# Autodesk Inventor assembly: Matchboxscope_VCM_v1
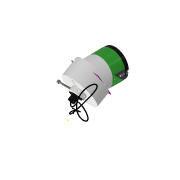
[picture p0: Inventor's stored thumbnail of the model, 180x180]
Saved by Autodesk Inventor 2022 (Build 260153000, 153)
## iProperties
Created: 2022-04-02
Part Number: Matchboxscope_VCM_v1
Document SubType Name: Assembly
Designer: Prakash Lab
Author: Prakash Lab
## Documents named in this file (13)
- C:\Users\diederichbenedict\Dropbox\Dokumente\Promotion\PROJECTS\Matchboxscope\INVENTOR\RELEASE\ESPECTROMETER\Workspace\Spectroscope_v0.iam
- C:\Users\diederichbenedict\Dropbox\Dokumente\Promotion\PROJECTS\Matchboxscope\INVENTOR\RELEASE\ESPECTROMETER\Workspace\00_ESP3-CAM.iam
- C:\Users\diederichbenedict\Dropbox\Dokumente\Promotion\PROJECTS\Matchboxscope\INVENTOR\RELEASE\ESPECTROMETER\Workspace\00_Powerbank.ipt
- C:\Users\diederichbenedict\Documents\Inventor\Content Center Files\R2022\de-DE\DIN 912\DIN 912 - M3 x 0.5 x 25 x 18.ipt
- C:\Users\diederichbenedict\Dropbox\Dokumente\Promotion\PROJECTS\Matchboxscope\INVENTOR\RELEASE\ESPECTROMETER\Workspace\Spectrometer_gratingholder_v0.ipt
- C:\Users\diederichbenedict\Dropbox\Dokumente\Promotion\PROJECTS\Matchboxscope\INVENTOR\RELEASE\ESPECTROMETER\Workspace\00_Grating_1000linesPerMM.ipt
- C:\Users\diederichbenedict\Dropbox\Dokumente\Promotion\PROJECTS\Matchboxscope\INVENTOR\RELEASE\ESPECTROMETER\Workspace\Spectrometer_pinholeholder_v0.ipt
- C:\Users\diederichbenedict\Dropbox\Dokumente\Promotion\PROJECTS\Matchboxscope\INVENTOR\RELEASE\InjectionMolded\00_mk8_nozzle_0.4STEP.ipt
- C:\Users\diederichbenedict\Dropbox\Dokumente\Promotion\PROJECTS\Matchboxscope\INVENTOR\RELEASE\ESPECTROMETER\Workspace\00_toslink_launcher_v3.ipt
- C:\Users\diederichbenedict\Dropbox\Dokumente\Promotion\PROJECTS\Matchboxscope\INVENTOR\RELEASE\ESPECTROMETER\Workspace\00_Toslink.ipt
- C:\Users\diederichbenedict\Dropbox\Dokumente\Promotion\PROJECTS\Matchboxscope\INVENTOR\RELEASE\InjectionMolded\IM_Matchboxscope_base.ipt
- C:\Users\diederichbenedict\Dropbox\Dokumente\Promotion\PROJECTS\Matchboxscope\INVENTOR\RELEASE\InjectionMolded\IM_Matchboxscope_plate.ipt
- C:\Users\diederichbenedict\Documents\Inventor\Content Center Files\R2022\de-DE\DIN 912\DIN 912 - M3 x 0.5 x 10 x 8.75.ipt
## Components (16 placed, 12 different names)
1. 00_ESP3-CAM:1 [sub-assembly]
2. 00_Powerbank:1
3. DIN 912 - ersetzt durch DIN EN ISO 4762 M3 x 25:4
4. DIN 912 - ersetzt durch DIN EN ISO 4762 M3 x 25:5
5. DIN 912 - ersetzt durch DIN EN ISO 4762 M3 x 25:6
6. DIN 912 - ersetzt durch DIN EN ISO 4762 M3 x 25:7
7. Spectrometer_gratingholder_v0:1 — Tangential:1, Einfügen:8
8. 00_Grating_1000linesPerMM:1 — Tangential:1, Fluchtend:5
9. Spectrometer_pinholeholder_v0:1 — Fluchtend:5, Einfügen:2
10. 00_mk8_nozzle_0.4STEP:1 — Einfügen:2, Einfügen:3
11. 00_toslink_launcher_v3:1 — Einfügen:3, Einfügen:4, Passend:6
12. 00_Toslink:1 — Einfügen:4
13. DIN 912 - ersetzt durch DIN EN ISO 4762 M3 x 25:8 — Passend:6
14. IM_Matchboxscope_base:1 — Einfügen:8, Einfügen:9
15. IM_Matchboxscope_plate:1 — Einfügen:9
16. DIN 912 - ersetzt durch DIN EN ISO 4762 M3 x 10:1
## Relationships (11: Insert 8, Tangent 1, Flush 1, Mate 1)
- Tangential:1 (-2 mm): Spectrometer_gratingholder_v0:1 ↔ 00_Grating_1000linesPerMM:1
- Fluchtend:5 [Flush]: 00_Grating_1000linesPerMM:1 ↔ Spectrometer_pinholeholder_v0:1
- Einfügen:2 [Insert]: Spectrometer_pinholeholder_v0:1 ↔ 00_mk8_nozzle_0.4STEP:1
- Einfügen:3 [Insert]: 00_mk8_nozzle_0.4STEP:1 ↔ 00_toslink_launcher_v3:1
- Einfügen:4 [Insert]: 00_toslink_launcher_v3:1 ↔ 00_Toslink:1
- Passend:6 [Mate]: 00_toslink_launcher_v3:1 ↔ DIN 912 - ersetzt durch DIN EN ISO 4762 M3 x 25:8
- [Insert]: IM_Matchboxscope_base:1 ↔ IM_Matchboxscope_plate:1
- [Insert]: IM_Matchboxscope_base:1 ↔ IM_Matchboxscope_plate:1
- [Insert] (-4 mm): IM_Matchboxscope_plate:1 ↔ DIN 912 - ersetzt durch DIN EN ISO 4762 M3 x 10:1
- Einfügen:8 [Insert]: Spectrometer_gratingholder_v0:1 ↔ IM_Matchboxscope_base:1
- Einfügen:9 [Insert]: IM_Matchboxscope_base:1 ↔ IM_Matchboxscope_plate:1
## Named parameters: d53_d45 = 0 mm, d54_d46 = 0 mm
